# Autodesk Inventor assembly: BakeBrakesAssembly
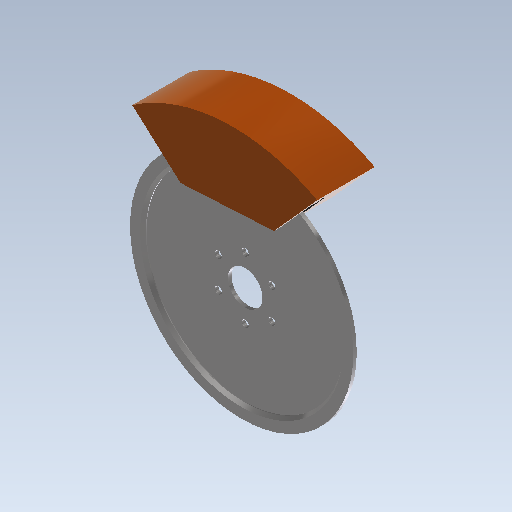
[picture p0: Inventor's stored thumbnail of the model, 512x512]
Saved by Autodesk Inventor 2021 (Build 250183000, 183)
## iProperties
Created: 2020-10-08
Part Number: BakeBrakesAssembly
Document SubType Name: Assembly
Designer: Federico
Author: Federico
## Documents named in this file (3)
- D:\Uni y2\Sem2\236\Design Project\Assembly 4\assembly 4-20201020T195157Z-001\assembly 4\BakeBrakesAssembly.iam
- D:\Uni y2\Sem2\236\Design Project\Assembly 4\assembly 4-20201020T195157Z-001\assembly 4\Calliper.ipt
- D:\Uni y2\Sem2\236\Design Project\Assembly 4\assembly 4-20201020T195157Z-001\assembly 4\DiskForBrakes.ipt
## Components (2 placed, 2 different names)
1. Calliper:1 — Rotational:1
2. DiskForBrakes:1 — Rotational:1
## Relationships (1: RevoluteJoint 1)
- Rotational:1 [RevoluteJoint]: Calliper:1 ↔ DiskForBrakes:1
